# Autodesk Inventor assembly: Connect_u2020_asm
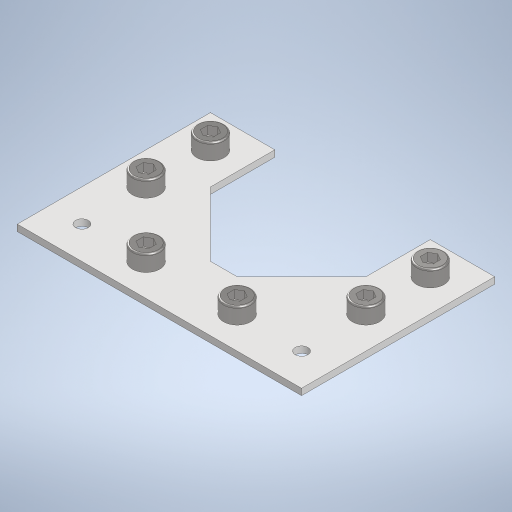
[picture p0: Inventor's stored thumbnail of the model, 512x512]
Saved by Autodesk Inventor 2024 (Build 280153000, 153)
## iProperties
Created: 2025-12-19
Part Number: Connect_u2020_asm
Document SubType Name: Assembly
Designer: schar
Author: schar
## Documents named in this file (4)
- C:\Users\schar\Desktop\projectBlueprint\AMSTS\hardware\Connect_u2020_asm.iam
- C:\Users\schar\Desktop\projectBlueprint\AMSTS\hardware\Connect_u2020.ipt
- C:\Users\schar\Desktop\projectBlueprint\AMSTS\hardware\tnut_m5_2020.ipt
- C:\Users\schar\Documents\Inventor\Content Center Files\R2024\en-US\ISO 4762(1)\DIN EN ISO 4762 - M5 x 8.ipt
## Components (13 placed, 3 different names)
1. Connect_u2020:1 — Mate:19, Mate:20, Mate:21, Mate:22, Mate:23, Mate:24, Mate:25, Mate:26, Mate:27, Mate:28, Mate:29, Mate:30, Mate:31, Mate:32, Rotational:1, Rotational:2, Rotational:3, Rotational:4, Rotational:5, Rotational:6
2. tnut_m5_2020:1 — Rotational:4
3. tnut_m5_2020:2 — Rotational:3
4. tnut_m5_2020:3 — Rotational:1
5. tnut_m5_2020:4 — Rotational:2
6. tnut_m5_2020:5 — Mate:20, Rotational:5
7. tnut_m5_2020:6 — Mate:19, Rotational:6
8. DIN EN ISO 4762 M5 x 8:1 — Mate:21, Mate:26
9. DIN EN ISO 4762 M5 x 8:2 — Mate:22, Mate:27
10. DIN EN ISO 4762 M5 x 8:3 — Mate:23, Mate:28
11. DIN EN ISO 4762 M5 x 8:4 — Mate:24, Mate:29
12. DIN EN ISO 4762 M5 x 8:5 — Mate:25, Mate:30
13. DIN EN ISO 4762 M5 x 8:6 — Mate:31, Mate:32
## Relationships (20: Mate 14, RevoluteJoint 6)
- Mate:19 (0.159 mm): Connect_u2020:1 ↔ tnut_m5_2020:6
- Mate:20 (0.159 mm): Connect_u2020:1 ↔ tnut_m5_2020:5
- Mate:21: Connect_u2020:1 ↔ DIN EN ISO 4762 M5 x 8:1
- Mate:22: Connect_u2020:1 ↔ DIN EN ISO 4762 M5 x 8:2
- Mate:23: Connect_u2020:1 ↔ DIN EN ISO 4762 M5 x 8:3
- Mate:24: Connect_u2020:1 ↔ DIN EN ISO 4762 M5 x 8:4
- Mate:25: Connect_u2020:1 ↔ DIN EN ISO 4762 M5 x 8:5
- Mate:26: Connect_u2020:1 ↔ DIN EN ISO 4762 M5 x 8:1
- Mate:27: Connect_u2020:1 ↔ DIN EN ISO 4762 M5 x 8:2
- Mate:28: Connect_u2020:1 ↔ DIN EN ISO 4762 M5 x 8:3
- Mate:29: Connect_u2020:1 ↔ DIN EN ISO 4762 M5 x 8:4
- Mate:30: Connect_u2020:1 ↔ DIN EN ISO 4762 M5 x 8:5
- Mate:31: Connect_u2020:1 ↔ DIN EN ISO 4762 M5 x 8:6
- Mate:32: Connect_u2020:1 ↔ DIN EN ISO 4762 M5 x 8:6
- Rotational:1 [RevoluteJoint] (0.159 mm): Connect_u2020:1 ↔ tnut_m5_2020:3
- Rotational:2 [RevoluteJoint] (0.159 mm): Connect_u2020:1 ↔ tnut_m5_2020:4
- Rotational:3 [RevoluteJoint] (0.159 mm): Connect_u2020:1 ↔ tnut_m5_2020:2
- Rotational:4 [RevoluteJoint] (0.159 mm): Connect_u2020:1 ↔ tnut_m5_2020:1
- Rotational:5 [RevoluteJoint] (0.159 mm): Connect_u2020:1 ↔ tnut_m5_2020:5
- Rotational:6 [RevoluteJoint] (0.159 mm): Connect_u2020:1 ↔ tnut_m5_2020:6
